# Autodesk Inventor assembly: АКБ Сборка
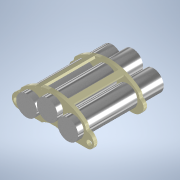
[picture p0: Inventor's stored thumbnail of the model, 180x180]
Saved by Autodesk Inventor 2022 (Build 260153000, 153)
## iProperties
Created: 2022-05-03
Part Number: АКБ Сборка
Document SubType Name: Assembly
Designer: Кочетов.А.И.
Author: Кочетов.А.И.
## Documents named in this file (5)
- C:\Users\BornO\Desktop\Отсек электроники v0.1 ТТ-1\АКБ\АКБ Сборка.iam
- C:\Users\BornO\Desktop\Отсек электроники v0.1 ТТ-1\АКБ\Крепление АКБ.ipt
- C:\Users\BornO\Desktop\Отсек электроники v0.1 ТТ-1\АКБ\Крепление АКБ нижнее.ipt
- C:\Users\BornO\Desktop\Отсек электроники v0.1 ТТ-1\АКБ\18650.ipt
- C:\Users\BornO\Desktop\Отсек электроники v0.1 ТТ-1\АКБ\АКБ Балка.ipt
## Components (8 placed, 4 different names)
1. Крепление АКБ:1 — Совмещение:3, Совмещение:4, Совмещение:5, Совмещение:6, Совмещение:7, Совмещение:8, Заподлицо:5
2. Крепление АКБ нижнее:1 — Совмещение:1, Совмещение:2, Заподлицо:1, Совмещение:3, Совмещение:4, Заподлицо:2, Заподлицо:3, Заподлицо:6, Совмещение:9, Совмещение:10, Совмещение:11, Совмещение:12, Совмещение:13, Заподлицо:7
3. 18650:1 — Совмещение:13, Заподлицо:7, Заподлицо:8, Заподлицо:9
4. 18650:2 — Совмещение:12, Заподлицо:8
5. 18650:3 — Совмещение:11, Заподлицо:9
6. АКБ Балка:1 — Заподлицо:3, Совмещение:7, Совмещение:8
7. АКБ Балка:2 — Заподлицо:6, Совмещение:9, Совмещение:10
8. АКБ Балка:3 — Совмещение:5, Совмещение:6, Заподлицо:2, Заподлицо:5
## Relationships (21: Mate 13, Flush 8)
- Совмещение:1 [Mate]: Крепление АКБ нижнее:1
- Совмещение:2 [Mate]: Крепление АКБ нижнее:1
- Заподлицо:1 [Flush]: Крепление АКБ нижнее:1
- Совмещение:3 [Mate]: Крепление АКБ:1 ↔ Крепление АКБ нижнее:1
- Совмещение:4 [Mate]: Крепление АКБ:1 ↔ Крепление АКБ нижнее:1
- Совмещение:5 [Mate]: Крепление АКБ:1 ↔ АКБ Балка:3
- Совмещение:6 [Mate]: Крепление АКБ:1 ↔ АКБ Балка:3
- Заподлицо:2 [Flush]: Крепление АКБ нижнее:1 ↔ АКБ Балка:3
- Заподлицо:3 [Flush]: Крепление АКБ нижнее:1 ↔ АКБ Балка:1
- Совмещение:7 [Mate]: Крепление АКБ:1 ↔ АКБ Балка:1
- Совмещение:8 [Mate]: Крепление АКБ:1 ↔ АКБ Балка:1
- Заподлицо:5 [Flush]: Крепление АКБ:1 ↔ АКБ Балка:3
- Заподлицо:6 [Flush]: Крепление АКБ нижнее:1 ↔ АКБ Балка:2
- Совмещение:9 [Mate]: Крепление АКБ нижнее:1 ↔ АКБ Балка:2
- Совмещение:10 [Mate]: Крепление АКБ нижнее:1 ↔ АКБ Балка:2
- Совмещение:11 [Mate]: Крепление АКБ нижнее:1 ↔ 18650:3
- Совмещение:12 [Mate]: Крепление АКБ нижнее:1 ↔ 18650:2
- Совмещение:13 [Mate]: Крепление АКБ нижнее:1 ↔ 18650:1
- Заподлицо:7 [Flush] (-5 mm): Крепление АКБ нижнее:1 ↔ 18650:1
- Заподлицо:8 [Flush]: 18650:1 ↔ 18650:2
- Заподлицо:9 [Flush]: 18650:1 ↔ 18650:3
